# Autodesk Inventor assembly: SyringeConcept1
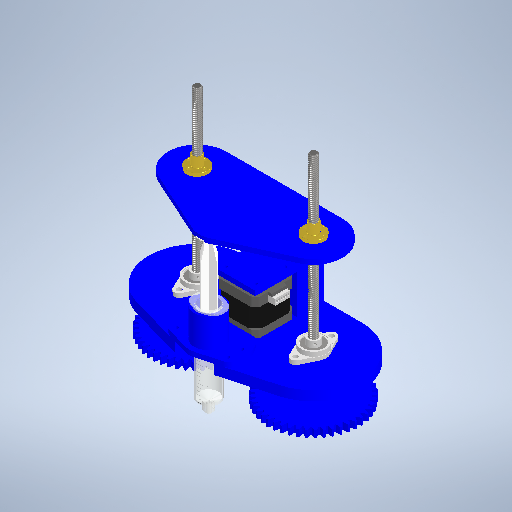
[picture p0: Inventor's stored thumbnail of the model, 512x512]
Saved by Autodesk Inventor 2025.2 (Build 292293000, 293)
## iProperties
Created: 2025-05-30
Part Number: SyringeConcept1
Document SubType Name: Assembly
Designer: Simon
Author: Simon
## Documents named in this file (16)
- C:\Users\Simon\Projects\Hydrogel-3D-Printer\Hardware\Bioprinter Machine Design\Extruder Concept 1\SyringeConcept1.iam
- C:\Users\Simon\Projects\Hydrogel-3D-Printer\Hardware\Bioprinter Machine Design\PartsFolder\Syringe\Rubber tampon_20ml.ipt
- C:\Users\Simon\Projects\Hydrogel-3D-Printer\Hardware\Bioprinter Machine Design\PartsFolder\Syringe\Syringe_cylinder_20ml.ipt
- C:\Users\Simon\Projects\Hydrogel-3D-Printer\Hardware\Bioprinter Machine Design\PartsFolder\Syringe\Syringe_piston_20ml.ipt
- C:\Users\Simon\Projects\Hydrogel-3D-Printer\Hardware\Bioprinter Machine Design\Extruder Concept 1\SyringePushMount.ipt
- C:\Users\Simon\Projects\Hydrogel-3D-Printer\Hardware\Bioprinter Machine Design\Extruder Concept 1\TR8x8-4_LeadScrew_200mm.ipt
- C:\Users\Simon\Projects\Hydrogel-3D-Printer\Hardware\Bioprinter Machine Design\PartsFolder\TR8x8-4_Nut.ipt
- C:\Users\Simon\Projects\Hydrogel-3D-Printer\Hardware\Bioprinter Machine Design\PartsFolder\Stepper_17HS4401.ipt
- C:\Users\Simon\Projects\Hydrogel-3D-Printer\Hardware\Bioprinter Machine Design\Extruder Concept 1\SyringeConcept1\Design Accelerator\Spur Gears2.iam
- C:\Users\Simon\Projects\Hydrogel-3D-Printer\Hardware\Bioprinter Machine Design\Extruder Concept 1\SpurGearPrimary.ipt
- C:\Users\Simon\Projects\Hydrogel-3D-Printer\Hardware\Bioprinter Machine Design\Extruder Concept 1\SpurGearSecondary.ipt
- C:\Users\Simon\Projects\Hydrogel-3D-Printer\Hardware\Bioprinter Machine Design\PartsFolder\Rigid Coupling 5,8\Rigid Coupling 5,8.iam
- C:\Users\Simon\Projects\Hydrogel-3D-Printer\Hardware\Bioprinter Machine Design\PartsFolder\Rigid Coupling 8,8.ipt
- C:\Users\Simon\Projects\Hydrogel-3D-Printer\Hardware\Bioprinter Machine Design\PartsFolder\Pillow Block Bearing 1\Zinc Alloy Pillow Block Flange Bearing KFL08 ID-8mm.iam
- C:\Users\Simon\Projects\Hydrogel-3D-Printer\Hardware\Bioprinter Machine Design\Extruder Concept 1\ExtruderFrame.ipt
- C:\Users\Simon\Projects\Hydrogel-3D-Printer\Hardware\Bioprinter Machine Design\Extruder Concept 1\SyringeHolder.ipt
## Components (20 placed, 15 different names)
1. Rubber tampon_20ml:1 — Mate:1, Mate:2
2. Syringe_cylinder_20ml:1 — Mate:3, Mate:28, Mate:39, Mate:41
3. Syringe_piston_20ml:1 — Mate:1, Mate:2, Mate:3, Mate:12
4. SyringePushMount:1 — Mate:4, Mate:5, Mate:6, Mate:7, Mate:8, Mate:9, Mate:10, Mate:12, Angle:1, Mate:28
5. TR8x8-4_LeadScrew_200mm:1 — Mate:13, Flush:1, Mate:15, Rotation:1, Mate:26, Mate:31
6. TR8x8-4_LeadScrew_200mm:2 — Mate:14, Flush:1, Mate:16, Rotation:2, Mate:25, Mate:27, Mate:32
7. TR8x8-4_Nut:1 — Mate:5, Mate:7, Mate:9, Mate:13
8. TR8x8-4_Nut:2 — Mate:6, Mate:8, Mate:10, Mate:14
9. Stepper_17HS4401:1 — Mate:17, Mate:20, Mate:21, Angle:1, Mate:38
10. Spur Gears:1 [sub-assembly]
11. Spur Gear1:1 — Flush:3, Mate:17, Mate:18, Mate:19, Rotation:3, Mate:22
12. Spur Gear2:1 — Mate:16, Flush:2, Flush:3, Mate:19, Rotation:2, Mate:24, Flush:5, Mate:25, Mate:29
13. Spur Gear2:2 — Mate:15, Flush:2, Mate:18, Rotation:1, Rotation:3, Mate:23
14. Rigid Coupling 5,8:1 [sub-assembly] — Mate:20, Mate:21, Mate:22, Mate:30
15. Rigid Coupling 8,8:1 — Mate:23, Flush:4
16. Rigid Coupling 8,8:2 — Mate:24, Flush:4, Flush:5
17. Zinc Alloy Pillow Block Flange Bearing KFL08 ID-8mm:1 [sub-assembly] — Mate:26, Flush:6, Mate:35, Mate:36, Mate:37
18. Zinc Alloy Pillow Block Flange Bearing KFL08 ID-8mm:2 [sub-assembly] — Mate:27, Flush:6, Mate:33, Mate:34
19. ExtruderFrame:1 — Mate:30, Mate:31, Mate:32, Mate:33, Mate:34, Mate:35, Mate:36, Mate:37, Mate:38, Mate:40, Mate:42, Mate:43, Mate:44
20. SyringeHolder:1 — Mate:39, Mate:40, Mate:41, Mate:42, Mate:43, Mate:44
## Relationships (53: Mate 43, Flush 6, RelateRotation 3, Angle 1)
- Mate:1: Rubber tampon_20ml:1 ↔ Syringe_piston_20ml:1
- Mate:2: Rubber tampon_20ml:1 ↔ Syringe_piston_20ml:1
- Mate:3: Syringe_cylinder_20ml:1 ↔ Syringe_piston_20ml:1
- Mate:4: SyringePushMount:1
- Mate:5: SyringePushMount:1 ↔ TR8x8-4_Nut:1
- Mate:6: SyringePushMount:1 ↔ TR8x8-4_Nut:2
- Mate:7: SyringePushMount:1 ↔ TR8x8-4_Nut:1
- Mate:8: SyringePushMount:1 ↔ TR8x8-4_Nut:2
- Mate:9: SyringePushMount:1 ↔ TR8x8-4_Nut:1
- Mate:10: SyringePushMount:1 ↔ TR8x8-4_Nut:2
- Mate:12: Syringe_piston_20ml:1 ↔ SyringePushMount:1
- Mate:13: TR8x8-4_LeadScrew_200mm:1 ↔ TR8x8-4_Nut:1
- Mate:14: TR8x8-4_LeadScrew_200mm:2 ↔ TR8x8-4_Nut:2
- Flush:1: TR8x8-4_LeadScrew_200mm:1 ↔ TR8x8-4_LeadScrew_200mm:2
- Mate:15: TR8x8-4_LeadScrew_200mm:1 ↔ Spur Gear2:2
- Mate:16: TR8x8-4_LeadScrew_200mm:2 ↔ Spur Gear2:1
- Flush:2: Spur Gear2:1 ↔ Spur Gear2:2
- Flush:3: Spur Gear1:1 ↔ Spur Gear2:1
- Mate:17: Stepper_17HS4401:1 ↔ Spur Gear1:1
- Mate:18 (60 mm): Spur Gear1:1 ↔ Spur Gear2:2
- Mate:19 (60 mm): Spur Gear1:1 ↔ Spur Gear2:1
- Rotation:1 [RelateRotation] (1 ul): TR8x8-4_LeadScrew_200mm:1 ↔ Spur Gear2:2
- Rotation:2 [RelateRotation] (1 ul): TR8x8-4_LeadScrew_200mm:2 ↔ Spur Gear2:1
- Rotation:3 [RelateRotation] (3 ul): Spur Gear1:1 ↔ Spur Gear2:2
- Mate:20: Stepper_17HS4401:1 ↔ Rigid Coupling 5,8:1
- Mate:21: Stepper_17HS4401:1 ↔ Rigid Coupling 5,8:1
- Mate:22: Spur Gear1:1 ↔ Rigid Coupling 5,8:1
- Angle:1 (90 deg): SyringePushMount:1 ↔ Stepper_17HS4401:1
- Mate:23: Spur Gear2:2 ↔ Rigid Coupling 8,8:1
- Mate:24: Spur Gear2:1 ↔ Rigid Coupling 8,8:2
- Flush:4: Rigid Coupling 8,8:1 ↔ Rigid Coupling 8,8:2
- Flush:5 (-12.5 mm): Spur Gear2:1 ↔ Rigid Coupling 8,8:2
- Mate:25: TR8x8-4_LeadScrew_200mm:2 ↔ Spur Gear2:1
- Mate:26: TR8x8-4_LeadScrew_200mm:1 ↔ Zinc Alloy Pillow Block Flange Bearing KFL08 ID-8mm:1
- Mate:27: TR8x8-4_LeadScrew_200mm:2 ↔ Zinc Alloy Pillow Block Flange Bearing KFL08 ID-8mm:2
- Flush:6: Zinc Alloy Pillow Block Flange Bearing KFL08 ID-8mm:1 ↔ Zinc Alloy Pillow Block Flange Bearing KFL08 ID-8mm:2
- Mate:28: Syringe_cylinder_20ml:1 ↔ SyringePushMount:1
- Mate:29: Spur Gear2:1
- Mate:30: Rigid Coupling 5,8:1 ↔ ExtruderFrame:1
- Mate:31: TR8x8-4_LeadScrew_200mm:1 ↔ ExtruderFrame:1
- Mate:32: TR8x8-4_LeadScrew_200mm:2 ↔ ExtruderFrame:1
- Mate:33: Zinc Alloy Pillow Block Flange Bearing KFL08 ID-8mm:2 ↔ ExtruderFrame:1
- Mate:34: Zinc Alloy Pillow Block Flange Bearing KFL08 ID-8mm:2 ↔ ExtruderFrame:1
- Mate:35: Zinc Alloy Pillow Block Flange Bearing KFL08 ID-8mm:1 ↔ ExtruderFrame:1
- Mate:36: Zinc Alloy Pillow Block Flange Bearing KFL08 ID-8mm:1 ↔ ExtruderFrame:1
- Mate:37: Zinc Alloy Pillow Block Flange Bearing KFL08 ID-8mm:1 ↔ ExtruderFrame:1
- Mate:38: Stepper_17HS4401:1 ↔ ExtruderFrame:1
- Mate:39: Syringe_cylinder_20ml:1 ↔ SyringeHolder:1
- Mate:40: ExtruderFrame:1 ↔ SyringeHolder:1
- Mate:41: Syringe_cylinder_20ml:1 ↔ SyringeHolder:1
- Mate:42: ExtruderFrame:1 ↔ SyringeHolder:1
- Mate:43: ExtruderFrame:1 ↔ SyringeHolder:1
- Mate:44: ExtruderFrame:1 ↔ SyringeHolder:1
